# Autodesk Inventor assembly: SEG soporte Trigger DC
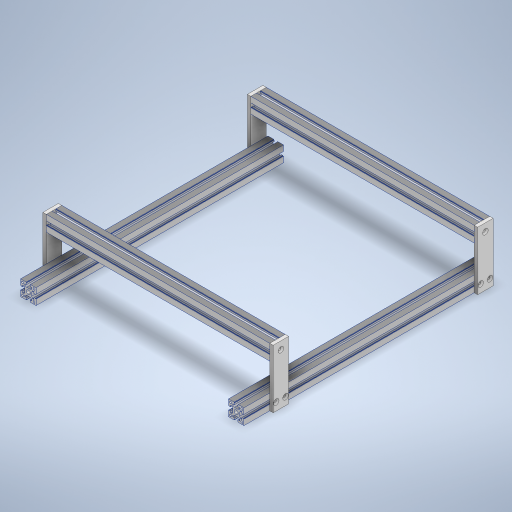
[picture p0: Inventor's stored thumbnail of the model, 512x512]
Saved by Autodesk Inventor 2024.2 (Build 282272000, 272)
## iProperties
Created: 2026-07-03
Part Number: SEG soporte Trigger DC
Document SubType Name: Assembly
Designer: ja.restrepo1
Author: ja.restrepo1
## Documents named in this file (6)
- I:\MICROMECANICA\ALTAS ENERGIAS\Deteccion de Muones\Detectores centelladores\Partes Detector Centellador\SE Base Trigger centellador\SEG soporte Trigger DC.iam
- I:\MICROMECANICA\ALTAS ENERGIAS\Deteccion de Muones\Detectores centelladores\Partes Detector Centellador\SE Base Trigger centellador\Caja Trigger DC.ipt
- I:\MICROMECANICA\ALTAS ENERGIAS\Deteccion de Muones\Detectores centelladores\Partes Detector Centellador\SE Base Trigger centellador\Soporte P45X45 largo.ipt
- I:\MICROMECANICA\ALTAS ENERGIAS\Deteccion de Muones\Detectores centelladores\Partes Detector Centellador\SE Base Trigger centellador\Prensa P45X45 Trigger.ipt
- I:\MICROMECANICA\ALTAS ENERGIAS\Deteccion de Muones\Detectores centelladores\Partes Detector Centellador\SE Base Trigger centellador\Sujetador prensa Trigger.ipt
- I:\MICROMECANICA\ALTAS ENERGIAS\Deteccion de Muones\Detectores centelladores\Partes Detector Centellador\SE Base Trigger centellador\Sujetador prensa Trigger_MIR.ipt
## Components (9 placed, 5 different names)
1. Caja Trigger DC:1 — Flush:1, Flush:2, Flush:3, Mate:1, Mate:2, Mate:3, Flush:6, Flush:7, Mate:5, Flush:16, Flush:20
2. Soporte P45X45 largo:1 — Mate:2, Flush:6, Flush:19, Flush:20
3. Soporte P45X45 largo:2 — Mate:3, Flush:7, Mate:7, Flush:19
4. Prensa P45X45 Trigger:1 — Flush:13, Mate:5, Flush:15, Flush:16, Mate:6, Flush:17, Flush:18
5. Prensa P45X45 Trigger:2 — Flush:14, Flush:15, Mate:6
6. Sujetador prensa Trigger_MIR:1
7. Sujetador prensa Trigger_MIR:2
8. Sujetador prensa Trigger:1 — Mate:7, Flush:17, Flush:18
9. Sujetador prensa Trigger:2
## Component patterns: (2 elements, first: Sujetador prensa Trigger:1)
## Relationships (19: Flush 13, Mate 6)
- Flush:1: Caja Trigger DC:1
- Flush:2: Caja Trigger DC:1
- Flush:3: Caja Trigger DC:1
- Mate:1: Caja Trigger DC:1
- Mate:2: Caja Trigger DC:1 ↔ Soporte P45X45 largo:1
- Mate:3: Caja Trigger DC:1 ↔ Soporte P45X45 largo:2
- Flush:6: Caja Trigger DC:1 ↔ Soporte P45X45 largo:1
- Flush:7: Caja Trigger DC:1 ↔ Soporte P45X45 largo:2
- Flush:13: Prensa P45X45 Trigger:1
- Flush:14: Prensa P45X45 Trigger:2
- Mate:5: Caja Trigger DC:1 ↔ Prensa P45X45 Trigger:1
- Flush:15: Prensa P45X45 Trigger:1 ↔ Prensa P45X45 Trigger:2
- Flush:16 (50 mm): Caja Trigger DC:1 ↔ Prensa P45X45 Trigger:1
- Mate:6 (550 mm): Prensa P45X45 Trigger:1 ↔ Prensa P45X45 Trigger:2
- Mate:7: Soporte P45X45 largo:2 ↔ Sujetador prensa Trigger:1
- Flush:17: Prensa P45X45 Trigger:1 ↔ Sujetador prensa Trigger:1
- Flush:18: Prensa P45X45 Trigger:1 ↔ Sujetador prensa Trigger:1
- Flush:19: Soporte P45X45 largo:1 ↔ Soporte P45X45 largo:2
- Flush:20 (25 mm): Caja Trigger DC:1 ↔ Soporte P45X45 largo:1
